# Autodesk Inventor assembly: Sandbox
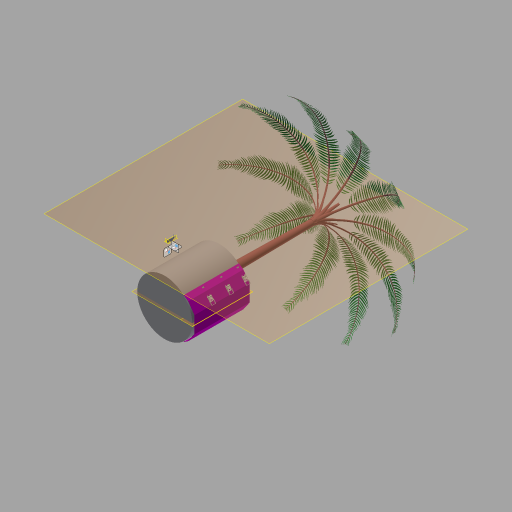
[picture p0: Inventor's stored thumbnail of the model, 512x512]
Saved by Autodesk Inventor 2023.2 (Build 272271000, 271)
## iProperties
Created: 2023-02-01
Part Number: Sandbox
Material: Generisch
Document SubType Name: Assembly
Designer: Raoul Messerli
Author: Raoul Messerli
## Documents named in this file (5)
- E:\GitHub\Pflanzenwagen\20_Inventor\40_Baugruppen\Sandbox.iam
- E:\GitHub\Pflanzenwagen\20_Inventor\10_Vorlage\Palme.iam
- E:\GitHub\Pflanzenwagen\20_Inventor\20_Einkaufteile\RatchetStrap\RatchetStrap\RatchetStrap.iam
- E:\GitHub\Pflanzenwagen\20_Inventor\30_Fertigungsteile\Blech1.ipt
- E:\GitHub\Pflanzenwagen\20_Inventor\20_Einkaufteile\RatchetStrap\Strap for Pflanzenwagen.ipt
## Components (6 placed, 4 different names)
1. Strap for Pflanzenwagen:1 — Passend:7, Passend:8, Fluchtend:9
2. Palme:1 [sub-assembly] — Fluchtend:1, Fluchtend:2, Tangential:1, Fluchtend:3, Fluchtend:4, Fluchtend:5
3. Blech1:1 — Fluchtend:1, Fluchtend:2, Tangential:1, Fluchtend:6, Passend:1, Passend:2, Passend:3, Fluchtend:7, Passend:4, Passend:5, Fluchtend:8, Passend:6
4. RatchetStrap:1 [sub-assembly] — Fluchtend:6, Passend:1, Passend:2
5. RatchetStrap:2 [sub-assembly] — Passend:3, Fluchtend:7, Passend:4
6. RatchetStrap:3 [sub-assembly] — Passend:5, Fluchtend:8, Passend:6
## Relationships (18: Flush 9, Mate 8, Tangent 1)
- Fluchtend:1 [Flush]: Palme:1 ↔ Blech1:1
- Fluchtend:2 [Flush]: Palme:1 ↔ Blech1:1
- Tangential:1: Palme:1 ↔ Blech1:1
- Fluchtend:3 [Flush]: Palme:1
- Fluchtend:4 [Flush]: Palme:1
- Fluchtend:5 [Flush]: Palme:1
- Fluchtend:6 [Flush]: Blech1:1 ↔ RatchetStrap:1
- Passend:1 [Mate]: Blech1:1 ↔ RatchetStrap:1
- Passend:2 [Mate]: Blech1:1 ↔ RatchetStrap:1
- Passend:3 [Mate]: Blech1:1 ↔ RatchetStrap:2
- Fluchtend:7 [Flush]: Blech1:1 ↔ RatchetStrap:2
- Passend:4 [Mate]: Blech1:1 ↔ RatchetStrap:2
- Passend:5 [Mate]: Blech1:1 ↔ RatchetStrap:3
- Fluchtend:8 [Flush]: Blech1:1 ↔ RatchetStrap:3
- Passend:6 [Mate]: Blech1:1 ↔ RatchetStrap:3
- Passend:7 [Mate]: Strap for Pflanzenwagen:1
- Passend:8 [Mate]: Strap for Pflanzenwagen:1
- Fluchtend:9 [Flush]: Strap for Pflanzenwagen:1
